# Autodesk Inventor assembly: IX
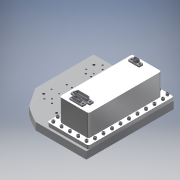
[picture p0: Inventor's stored thumbnail of the model, 180x180]
Saved by Autodesk Inventor 2017 (Build 210142000, 142)
## iProperties
Created: 2016-12-06
Part Number: IX
Document SubType Name: Assembly
Designer: qupec
Mass: 1513.48 g
Surface Area: 2866.97 cm^2
Volume: 582.995 cm^3
Density: 2.59604 g/cm^3
Author: qupec
## Documents named in this file (21)
- C:\UMD\BPP\ROCKSAT X\STAR\CAD\Mechanical\Exploded Views\IX.iam
- C:\UMD\BPP\ROCKSAT X\STAR\CAD\Mechanical\Full payload assembly\Subsystems\Electronics\Electronics Stack.iam
- C:\UMD\BPP\ROCKSAT X\STAR\CAD\Mechanical\Full payload assembly\Base Plate.ipt
- C:\UMD\BPP\ROCKSAT X\STAR\CAD\Mechanical\Full payload assembly\Subsystems\Electronics\Electronics Box.ipt
- C:\UMD\BPP\ROCKSAT X\STAR\CAD\Mechanical\Full payload assembly\Subsystems\Electronics\9pin female connector.ipt
- C:\UMD\BPP\ROCKSAT X\STAR\CAD\Mechanical\Full payload assembly\Subsystems\Electronics\31pin female connector.ipt
- C:\UMD\BPP\ROCKSAT X\STAR\CAD\Mechanical\Full payload assembly\Subsystems\Electronics\15pin female connector.ipt
- C:\UMD\BPP\ROCKSAT X\STAR\CAD\Mechanical\Full payload assembly\Subsystems\Fasteners\Num4 Narrow Split Washer.ipt
- C:\UMD\BPP\ROCKSAT X\STAR\CAD\Mechanical\Full payload assembly\Subsystems\Fasteners\4-40 .5in Socket Screw.ipt
- C:\UMD\BPP\ROCKSAT X\star\CAD\Mechanical\Subsystems\Full payload assembly mk 2\AIP\FEA\c3occb59c.fins
- C:\UMD\BPP\ROCKSAT X\star\CAD\Mechanical\Subsystems\Full payload assembly mk 2\AIP\FEA\c3occb5b4.fsat
- C:\UMD\BPP\ROCKSAT X\star\CAD\Mechanical\Subsystems\Full payload assembly mk 2\AIP\FEA\c3occb5b4.ftes
- C:\UMD\BPP\ROCKSAT X\star\CAD\Mechanical\Subsystems\Full payload assembly mk 2\AIP\FEA\c3occb5b4.fwiz
- C:\UMD\BPP\ROCKSAT X\star\CAD\Mechanical\Subsystems\Full payload assembly mk 2\AIP\FEA\c3occb5c0.fins
- C:\UMD\BPP\ROCKSAT X\star\CAD\Mechanical\Subsystems\Full payload assembly mk 2\AIP\FEA\c3occb5c0.fsat
- C:\UMD\BPP\ROCKSAT X\star\CAD\Mechanical\Subsystems\Full payload assembly mk 2\AIP\FEA\c3occb5c0.ftes
- C:\UMD\BPP\ROCKSAT X\star\CAD\Mechanical\Subsystems\Full payload assembly mk 2\AIP\FEA\c3occb5c0.fwiz
- C:\UMD\BPP\ROCKSAT X\star\CAD\Mechanical\Subsystems\Full payload assembly mk 2\AIP\FEA\c3occb60w.fmsh
- C:\UMD\BPP\ROCKSAT X\star\CAD\Mechanical\Subsystems\Full payload assembly mk 2\AIP\FEA\c3occb60x.fres
- C:\UMD\BPP\ROCKSAT X\star\CAD\Mechanical\Subsystems\Full payload assembly mk 2\AIP\FEA\c3occb6sg.fmsh
- C:\UMD\BPP\ROCKSAT X\star\CAD\Mechanical\Subsystems\Full payload assembly mk 2\AIP\FEA\c3occb6sh.fres
## Components (62 placed, 8 different names)
1. Electronics Stack:1 [sub-assembly] — Flush:41, Flush:42, Mate:397
2. Base Plate:1 — Mate:124, Flush:29, Flush:32, Mate:163, Flush:33, Flush:40, Mate:397
3. 31pin female connector:1 — Flush:34, Flush:35, Mate:164
4. 15pin female connector:1 — Mate:165, Flush:43, Flush:44
5. 9pin female connector:1 — Flush:38, Flush:39, Mate:166
6. Electronics Box:1 — Mate:163, Flush:33, Flush:34, Flush:35, Mate:164, Flush:38, Flush:39, Mate:165, Mate:166, Flush:40, Flush:41, Flush:42, Flush:43, Flush:44, Mate:400, Mate:401, Mate:402, Mate:403, Mate:404, Mate:405, Mate:406, Mate:407, Mate:408, Mate:409, Mate:410, Mate:411, Mate:412, Mate:413, Mate:414, Mate:415, Mate:416, Mate:417, Mate:418, Mate:419, Mate:420, Mate:421, Mate:422, Mate:423, Mate:424, Mate:425, Mate:426, Mate:427, Mate:428, Mate:429, Mate:430, Mate:431, Mate:432, Mate:433, Mate:434, Mate:435, Mate:437, Mate:438, Mate:439, Mate:440, Mate:441, Mate:442, Mate:443, Mate:444, Mate:445, Mate:446, Mate:447, Mate:448, Mate:449, Mate:450, Mate:451, Mate:452, Mate:453, Mate:454, Mate:455, Mate:456, Mate:457, Mate:458, Mate:459, Mate:518
7. Num4 Narrow Split Washer:1 — Mate:411, Mate:457, Mate:645
8. Num4 Narrow Split Washer:2 — Mate:413, Mate:419, Mate:455
9. Num4 Narrow Split Washer:3 — Mate:415, Mate:450
10. Num4 Narrow Split Washer:4 — Mate:414, Mate:444
11. Num4 Narrow Split Washer:5 — Mate:412, Mate:452
12. Num4 Narrow Split Washer:6 — Mate:410, Mate:443
13. Num4 Narrow Split Washer:7 — Mate:409, Mate:453
14. Num4 Narrow Split Washer:8 — Mate:408, Mate:441
15. Num4 Narrow Split Washer:9 — Mate:420, Mate:437
16. Num4 Narrow Split Washer:10 — Mate:423, Mate:451
17. Num4 Narrow Split Washer:11 — Mate:407, Mate:445
18. Num4 Narrow Split Washer:12 — Mate:405, Mate:447
19. Num4 Narrow Split Washer:13 — Mate:428, Mate:433
20. Num4 Narrow Split Washer:14 — Mate:426, Mate:435
21. Num4 Narrow Split Washer:15 — Mate:418, Mate:430
22. Num4 Narrow Split Washer:17 — Mate:422, Mate:454
23. Num4 Narrow Split Washer:18 — Mate:417, Mate:431
24. Num4 Narrow Split Washer:19 — Mate:425, Mate:456
25. Num4 Narrow Split Washer:20 — Mate:424, Mate:439
26. Num4 Narrow Split Washer:21 — Mate:427, Mate:434
27. Num4 Narrow Split Washer:22 — Mate:429, Mate:432
28. Num4 Narrow Split Washer:23 — Mate:421, Mate:438
29. Num4 Narrow Split Washer:24 — Mate:404, Mate:440
30. Num4 Narrow Split Washer:25 — Mate:401, Mate:442
31. Num4 Narrow Split Washer:26 — Mate:400, Mate:416, Mate:449
32. Num4 Narrow Split Washer:27 — Mate:402, Mate:406, Mate:446
33. Num4 Narrow Split Washer:28 — Mate:403, Mate:448
34. Num4 Narrow Split Washer:29 — Mate:458, Mate:459
35. 4-40 .5in Socket Screw:1
36. 4-40 .5in Socket Screw:2
37. 4-40 .5in Socket Screw:3
38. 4-40 .5in Socket Screw:4
39. 4-40 .5in Socket Screw:5
40. 4-40 .5in Socket Screw:6
41. 4-40 .5in Socket Screw:7
42. 4-40 .5in Socket Screw:8
43. 4-40 .5in Socket Screw:9
44. 4-40 .5in Socket Screw:10
45. 4-40 .5in Socket Screw:11
46. 4-40 .5in Socket Screw:12
47. 4-40 .5in Socket Screw:13
48. 4-40 .5in Socket Screw:14
49. 4-40 .5in Socket Screw:15 — Mate:518
50. 4-40 .5in Socket Screw:16
51. 4-40 .5in Socket Screw:17 — Mate:645
52. 4-40 .5in Socket Screw:18
53. 4-40 .5in Socket Screw:19
54. 4-40 .5in Socket Screw:20
55. 4-40 .5in Socket Screw:21
56. 4-40 .5in Socket Screw:22
57. 4-40 .5in Socket Screw:23
58. 4-40 .5in Socket Screw:24
59. 4-40 .5in Socket Screw:25
60. 4-40 .5in Socket Screw:26
61. 4-40 .5in Socket Screw:27
62. 4-40 .5in Socket Screw:28
## Relationships (134: Mate 122, Flush 12)
- Mate:124: Base Plate:1
- Flush:29: Base Plate:1
- Flush:32: Base Plate:1
- Mate:163: Base Plate:1 ↔ Electronics Box:1
- Flush:33: Base Plate:1 ↔ Electronics Box:1
- Flush:34 (12.7 mm): 31pin female connector:1 ↔ Electronics Box:1
- Flush:35 (6.35 mm): 31pin female connector:1 ↔ Electronics Box:1
- Mate:164: 31pin female connector:1 ↔ Electronics Box:1
- Flush:38 (6.35 mm): 9pin female connector:1 ↔ Electronics Box:1
- Flush:39 (-6.35 mm): 9pin female connector:1 ↔ Electronics Box:1
- Mate:165: 15pin female connector:1 ↔ Electronics Box:1
- Mate:166: 9pin female connector:1 ↔ Electronics Box:1
- Flush:40: Base Plate:1 ↔ Electronics Box:1
- Flush:41 (3.175 mm): Electronics Stack:1 ↔ Electronics Box:1
- Flush:42: Electronics Stack:1 ↔ Electronics Box:1
- Flush:43 (3.81 mm): 15pin female connector:1 ↔ Electronics Box:1
- Flush:44 (12.7 mm): 15pin female connector:1 ↔ Electronics Box:1
- Mate:397: Electronics Stack:1 ↔ Base Plate:1
- Mate:400: Electronics Box:1 ↔ Num4 Narrow Split Washer:26
- Mate:401: Electronics Box:1 ↔ Num4 Narrow Split Washer:25
- Mate:402: Electronics Box:1 ↔ Num4 Narrow Split Washer:27
- Mate:403: Electronics Box:1 ↔ Num4 Narrow Split Washer:28
- Mate:404: Electronics Box:1 ↔ Num4 Narrow Split Washer:24
- Mate:405: Electronics Box:1 ↔ Num4 Narrow Split Washer:12
- Mate:406: Electronics Box:1 ↔ Num4 Narrow Split Washer:27
- Mate:407: Electronics Box:1 ↔ Num4 Narrow Split Washer:11
- Mate:408: Electronics Box:1 ↔ Num4 Narrow Split Washer:8
- Mate:409: Electronics Box:1 ↔ Num4 Narrow Split Washer:7
- Mate:410: Electronics Box:1 ↔ Num4 Narrow Split Washer:6
- Mate:411: Electronics Box:1 ↔ Num4 Narrow Split Washer:1
- Mate:412: Electronics Box:1 ↔ Num4 Narrow Split Washer:5
- Mate:413: Electronics Box:1 ↔ Num4 Narrow Split Washer:2
- Mate:414: Electronics Box:1 ↔ Num4 Narrow Split Washer:4
- Mate:415: Electronics Box:1 ↔ Num4 Narrow Split Washer:3
- Mate:416: Electronics Box:1 ↔ Num4 Narrow Split Washer:26
- Mate:417: Electronics Box:1 ↔ Num4 Narrow Split Washer:18
- Mate:418: Electronics Box:1 ↔ Num4 Narrow Split Washer:15
- Mate:419: Electronics Box:1 ↔ Num4 Narrow Split Washer:2
- Mate:420: Electronics Box:1 ↔ Num4 Narrow Split Washer:9
- Mate:421: Electronics Box:1 ↔ Num4 Narrow Split Washer:23
- Mate:422: Electronics Box:1 ↔ Num4 Narrow Split Washer:17
- Mate:423: Electronics Box:1 ↔ Num4 Narrow Split Washer:10
- Mate:424: Electronics Box:1 ↔ Num4 Narrow Split Washer:20
- Mate:425: Electronics Box:1 ↔ Num4 Narrow Split Washer:19
- Mate:426: Electronics Box:1 ↔ Num4 Narrow Split Washer:14
- Mate:427: Electronics Box:1 ↔ Num4 Narrow Split Washer:21
- Mate:428: Electronics Box:1 ↔ Num4 Narrow Split Washer:13
- Mate:429: Electronics Box:1 ↔ Num4 Narrow Split Washer:22
- Mate:430: Electronics Box:1 ↔ Num4 Narrow Split Washer:15
- Mate:431: Electronics Box:1 ↔ Num4 Narrow Split Washer:18
- Mate:432: Electronics Box:1 ↔ Num4 Narrow Split Washer:22
- Mate:433: Electronics Box:1 ↔ Num4 Narrow Split Washer:13
- Mate:434: Electronics Box:1 ↔ Num4 Narrow Split Washer:21
- Mate:435: Electronics Box:1 ↔ Num4 Narrow Split Washer:14
- Mate:437: Electronics Box:1 ↔ Num4 Narrow Split Washer:9
- Mate:438: Electronics Box:1 ↔ Num4 Narrow Split Washer:23
- Mate:439: Electronics Box:1 ↔ Num4 Narrow Split Washer:20
- Mate:440: Electronics Box:1 ↔ Num4 Narrow Split Washer:24
- Mate:441: Electronics Box:1 ↔ Num4 Narrow Split Washer:8
- Mate:442: Electronics Box:1 ↔ Num4 Narrow Split Washer:25
- Mate:443: Electronics Box:1 ↔ Num4 Narrow Split Washer:6
- Mate:444: Electronics Box:1 ↔ Num4 Narrow Split Washer:4
- Mate:445: Electronics Box:1 ↔ Num4 Narrow Split Washer:11
- Mate:446: Electronics Box:1 ↔ Num4 Narrow Split Washer:27
- Mate:447: Electronics Box:1 ↔ Num4 Narrow Split Washer:12
- Mate:448: Electronics Box:1 ↔ Num4 Narrow Split Washer:28
- Mate:449: Electronics Box:1 ↔ Num4 Narrow Split Washer:26
- Mate:450: Electronics Box:1 ↔ Num4 Narrow Split Washer:3
- Mate:451: Electronics Box:1 ↔ Num4 Narrow Split Washer:10
- Mate:452: Electronics Box:1 ↔ Num4 Narrow Split Washer:5
- Mate:453: Electronics Box:1 ↔ Num4 Narrow Split Washer:7
- Mate:454: Electronics Box:1 ↔ Num4 Narrow Split Washer:17
- Mate:455: Electronics Box:1 ↔ Num4 Narrow Split Washer:2
- Mate:456: Electronics Box:1 ↔ Num4 Narrow Split Washer:19
- Mate:457: Electronics Box:1 ↔ Num4 Narrow Split Washer:1
- Mate:458: Electronics Box:1 ↔ Num4 Narrow Split Washer:29
- Mate:459: Electronics Box:1 ↔ Num4 Narrow Split Washer:29
- [Mate]: Num4 Narrow Split Washer:29 ↔ 4-40 .5in Socket Screw:13
- [Mate]: Num4 Narrow Split Washer:4 ↔ 4-40 .5in Socket Screw:5
- [Mate]: Num4 Narrow Split Washer:20 ↔ 4-40 .5in Socket Screw:4
- [Mate]: Num4 Narrow Split Washer:9 ↔ 4-40 .5in Socket Screw:26
- [Mate]: Num4 Narrow Split Washer:14 ↔ 4-40 .5in Socket Screw:1
- [Mate]: Num4 Narrow Split Washer:21 ↔ 4-40 .5in Socket Screw:11
- [Mate]: Num4 Narrow Split Washer:13 ↔ 4-40 .5in Socket Screw:2
- [Mate]: Num4 Narrow Split Washer:22 ↔ 4-40 .5in Socket Screw:23
- [Mate]: Num4 Narrow Split Washer:18 ↔ 4-40 .5in Socket Screw:22
- [Mate]: Num4 Narrow Split Washer:15 ↔ 4-40 .5in Socket Screw:28
- [Mate]: Num4 Narrow Split Washer:24 ↔ 4-40 .5in Socket Screw:16
- [Mate]: Num4 Narrow Split Washer:8 ↔ 4-40 .5in Socket Screw:14
- [Mate]: Num4 Narrow Split Washer:25 ↔ 4-40 .5in Socket Screw:15
- [Mate]: Num4 Narrow Split Washer:6 ↔ 4-40 .5in Socket Screw:24
- [Mate]: Num4 Narrow Split Washer:11 ↔ 4-40 .5in Socket Screw:9
- [Mate]: Num4 Narrow Split Washer:27 ↔ 4-40 .5in Socket Screw:21
- [Mate]: Num4 Narrow Split Washer:12 ↔ 4-40 .5in Socket Screw:18
- [Mate]: Num4 Narrow Split Washer:28 ↔ 4-40 .5in Socket Screw:19
- [Mate]: Num4 Narrow Split Washer:26 ↔ 4-40 .5in Socket Screw:20
- [Mate]: Num4 Narrow Split Washer:3 ↔ 4-40 .5in Socket Screw:25
- [Mate]: Num4 Narrow Split Washer:10 ↔ 4-40 .5in Socket Screw:8
- [Mate]: Num4 Narrow Split Washer:5 ↔ 4-40 .5in Socket Screw:10
- [Mate]: Num4 Narrow Split Washer:7 ↔ 4-40 .5in Socket Screw:7
- [Mate]: Num4 Narrow Split Washer:17 ↔ 4-40 .5in Socket Screw:3
- [Mate]: Num4 Narrow Split Washer:2 ↔ 4-40 .5in Socket Screw:12
- [Mate]: Num4 Narrow Split Washer:19 ↔ 4-40 .5in Socket Screw:6
- [Mate]: Num4 Narrow Split Washer:1 ↔ 4-40 .5in Socket Screw:17
- [Mate]: Electronics Box:1 ↔ 4-40 .5in Socket Screw:24
- [Mate]: Electronics Box:1 ↔ 4-40 .5in Socket Screw:14
- [Mate]: Electronics Box:1 ↔ 4-40 .5in Socket Screw:16
- [Mate]: Electronics Box:1 ↔ 4-40 .5in Socket Screw:28
- [Mate]: Electronics Box:1 ↔ 4-40 .5in Socket Screw:22
- [Mate]: Electronics Box:1 ↔ 4-40 .5in Socket Screw:23
- [Mate]: Electronics Box:1 ↔ 4-40 .5in Socket Screw:2
- [Mate]: Electronics Box:1 ↔ 4-40 .5in Socket Screw:11
- [Mate]: Num4 Narrow Split Washer:14 ↔ 4-40 .5in Socket Screw:1
- [Mate]: Num4 Narrow Split Washer:9 ↔ 4-40 .5in Socket Screw:26
- [Mate]: Num4 Narrow Split Washer:23 ↔ 4-40 .5in Socket Screw:27
- [Mate]: Electronics Box:1 ↔ 4-40 .5in Socket Screw:27
- [Mate]: Num4 Narrow Split Washer:20 ↔ 4-40 .5in Socket Screw:4
- [Mate]: Num4 Narrow Split Washer:4 ↔ 4-40 .5in Socket Screw:5
- [Mate]: Num4 Narrow Split Washer:29 ↔ 4-40 .5in Socket Screw:13
- [Mate]: Num4 Narrow Split Washer:11 ↔ 4-40 .5in Socket Screw:9
- [Mate]: Num4 Narrow Split Washer:27 ↔ 4-40 .5in Socket Screw:21
- [Mate]: Num4 Narrow Split Washer:12 ↔ 4-40 .5in Socket Screw:18
- [Mate]: Num4 Narrow Split Washer:28 ↔ 4-40 .5in Socket Screw:19
- [Mate]: Num4 Narrow Split Washer:26 ↔ 4-40 .5in Socket Screw:20
- [Mate]: Num4 Narrow Split Washer:3 ↔ 4-40 .5in Socket Screw:25
- [Mate]: Electronics Box:1 ↔ 4-40 .5in Socket Screw:8
- [Mate]: Electronics Box:1 ↔ 4-40 .5in Socket Screw:10
- [Mate]: Num4 Narrow Split Washer:7 ↔ 4-40 .5in Socket Screw:7
- [Mate]: Num4 Narrow Split Washer:17 ↔ 4-40 .5in Socket Screw:3
- [Mate]: Num4 Narrow Split Washer:2 ↔ 4-40 .5in Socket Screw:12
- [Mate]: Num4 Narrow Split Washer:19 ↔ 4-40 .5in Socket Screw:6
- [Mate]: Num4 Narrow Split Washer:29 ↔ 4-40 .5in Socket Screw:13
- Mate:518: Electronics Box:1 ↔ 4-40 .5in Socket Screw:15
- Mate:645: Num4 Narrow Split Washer:1 ↔ 4-40 .5in Socket Screw:17
## Named parameters: sa_3 = 0, sa_4 = 29260.8, sa_5 = 0, sa_6 = 6894.76
note: some values were not read from the file. Shown as the stored number, unit unknown: "sa_3", "sa_4", "sa_5", "sa_6".
